# Autodesk Inventor assembly: C-AFDF22-25
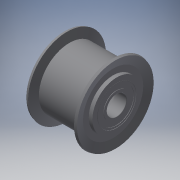
[picture p0: Inventor's stored thumbnail of the model, 180x180]
Saved by Autodesk Inventor 2019 (Build 230136000, 136)
## iProperties
Category: PARTsolutions
Company: MISUMI
Created: 2023-11-09
Part Number: C-AFDF22-25
Catalog Web Link: www.cadenas.de
Description: C-AFBD, C-AFDF-Economy Idlers Backside Tension Type
Vendor: MISUMI
Document SubType Name: Assembly
Designer: psAdmin
Manufacturer: MISUMI
Mass: 8.49496 g
Surface Area: 60.5331 cm^2
Volume: 8.49496 cm^3
Density: 1 g/cm^3
Title: C-AFDF22-25
Author: Cadenas PARTsolutions
Comments: Economy Idlers Backside Tension Type
PSOL_IDENT_0: {$CADENAS_DATA/23d-libs/misumi/metric/51_timing_pulleys/c_afbd_asmtab.prj},192 {VTYP=3D},{STYP=ASSTA
PSOL_IDENT_1: B},{NB=C-AFDF22-25},{LINA=C-AFDF22-25},{NN=C-AFBD, C-AFDF},{DATE=13.09.2022 06:49:12},{GEOMDATE=18.0
PSOL_IDENT_2: 5.2021 06:13:57},{VERSION=},{LINEID=100},{WBVAR=TS,TYPE},{WBNUMERIC=}  {NB=C-AFDF22-25},{LINA=C-AFDF
PSOL_IDENT_3: 22-25},{KT=DUMMY},{PN=C-AFDF22-25},{TS=BSB},{TSALG= 'CB','Center Bearing Type','BSB','Both Sides Bea
PSOL_IDENT_4: ring Type' },{TYPE=C-AFDF},{TYPEALG= 'C-AFBD','No Flange','C-AFDF','Flanged' },{W=22.0},{NOM=25},{D=
PSOL_IDENT_5: 25},{F=32},{A=17.0},{ABI=-},{ABM=150},{S=0.00},{NO=688ZZx2},{BN=6000},{DD=8},{B=5.0},{RR=-},{E=0.000
PSOL_IDENT_6: },{BD=0},{DH=0.000},{DD2=0},{RTT=0.000},{PTT=1.000},{CIF=0.000},{PPATH=c_afbd/c_afbd_asmtpl.prj}
NB: C-AFDF22-25
NN: C-AFBD, C-AFDF
NT: Economy Idlers Backside Tension Type
NBSYN: $PN.
LINA: C-AFDF22-25
CATALOG: Misumi
PN: C-AFDF22-25
TS: Both Sides Bearing Type
TYPE: Flanged
W: 22
NOM: 25
D: 25
F: 32
A: 17
ABI: -
ABM: 150
S: 0
NO: 688ZZx2
DD: 8
B: 5
RR: -
SUPPLIER: MISUMI
ARTICLENO: C-AFDF22-25
BOMINFO: C-AFDF22-25
CREATOR: CADENAS GmbH
## Documents named in this file (3)
- e:\temp\worker_COMMON_2\temp\tmp_3796_2_DHTH1\format_0\C-AFDF22-25.iam
- e:\temp\worker_COMMON_2\temp\tmp_3796_2_DHTH1\format_0\C-AFDF22-25_bw.ipt
- e:\temp\worker_COMMON_2\temp\tmp_3796_2_DHTH1\format_0\bearing_688.ipt
## Components (3 placed, 2 different names)
1. C-AFDF22-25_bw:1 — b600_1_XY@1 <-> to_housing_center_XY@2, b600_1_Z@1 <-> to_housing_center_Z@2, b600_1_YZ@1 <-> to_housing_center_YZ@2, b600_2_XY@1 <-> to_housing_center_XY@3, b600_2_Z@1 <-> to_housing_center_Z@3, b600_2_YZ@1 <-> to_housing_center_YZ@3
2. bearing_688:1 — b600_1_XY@1 <-> to_housing_center_XY@2, b600_1_Z@1 <-> to_housing_center_Z@2, b600_1_YZ@1 <-> to_housing_center_YZ@2
3. bearing_688:2 — b600_2_XY@1 <-> to_housing_center_XY@3, b600_2_Z@1 <-> to_housing_center_Z@3, b600_2_YZ@1 <-> to_housing_center_YZ@3
## Relationships (6: Mate 4, Angle 2)
- b600_1_XY@1 <-> to_housing_center_XY@2 [Mate]: C-AFDF22-25_bw:1 ↔ bearing_688:1
- b600_1_Z@1 <-> to_housing_center_Z@2 [Mate]: C-AFDF22-25_bw:1 ↔ bearing_688:1
- b600_1_YZ@1 <-> to_housing_center_YZ@2 [Angle] (0 deg): C-AFDF22-25_bw:1 ↔ bearing_688:1
- b600_2_XY@1 <-> to_housing_center_XY@3 [Mate]: C-AFDF22-25_bw:1 ↔ bearing_688:2
- b600_2_Z@1 <-> to_housing_center_Z@3 [Mate]: C-AFDF22-25_bw:1 ↔ bearing_688:2
- b600_2_YZ@1 <-> to_housing_center_YZ@3 [Angle] (0 deg): C-AFDF22-25_bw:1 ↔ bearing_688:2
